# Autodesk Inventor assembly: RR_ThreeWay-A
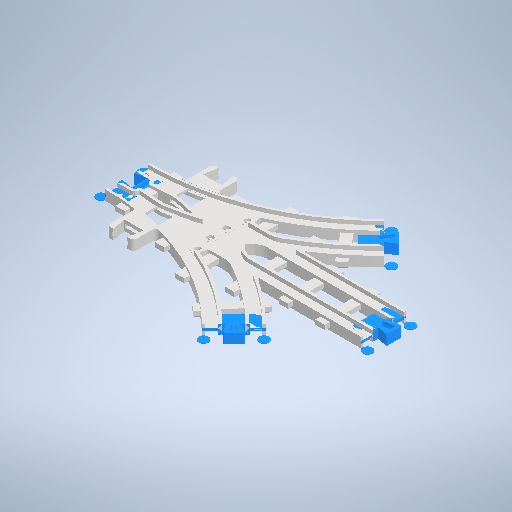
[picture p0: Inventor's stored thumbnail of the model, 512x512]
Saved by Autodesk Inventor 2025.1 (Build 291241000, 241)
## iProperties
Created: 2025-03-06
Part Number: RR_ThreeWay-A
Document SubType Name: Assembly
Designer: kumagai
Author: kumagai
## Documents named in this file (11)
- X:\Develop\CAD\PlaRails\RealRails\RR_ThreeWay.iam
- X:\Develop\CAD\PlaRails\Common\RailJointRS\FemaleDoubleSideWT.ipt
- X:\Develop\CAD\PlaRails\Common\RailJointRS.ipt
- X:\Develop\CAD\PlaRails\Common\RailJointRS\MaleDoubleSideWT.ipt
- X:\Develop\CAD\PlaRails\RealRails\RR_ThreeWay.ipt
- X:\Develop\CAD\PlaRails\RealRails\RR_ThreeWayPillow.ipt
- X:\Develop\CAD\PlaRails\RealRails\RR_ThreeWay\RR_ThreeWay-all.ipt
- RR_ThreeWay-A.iam
- RR_ThreeWay-AwoS.iam
- RR_ThreeWay-B.iam
- RR_ThreeWay-BwoS.iam
## Components (6 placed, 4 different names)
1. RR_ThreeWay-all:1 — フラッシュ:1, メイト:1, フラッシュ:2, フラッシュ:3, メイト:2, フラッシュ:4, フラッシュ:5, メイト:3, フラッシュ:6, フラッシュ:7, メイト:4, フラッシュ:8
2. FemaleDoubleSideWT:1 — フラッシュ:1, メイト:1, フラッシュ:2
3. MaleDoubleSideWT:2 — フラッシュ:3, メイト:2, フラッシュ:4
4. MaleDoubleSideWT:3 — フラッシュ:5, メイト:3, フラッシュ:6
5. RR_ThreeWayPillow:1
6. MaleDoubleSideWT:4 — フラッシュ:7, メイト:4, フラッシュ:8
## Relationships (12: Flush 8, Mate 4)
- フラッシュ:1 [Flush]: RR_ThreeWay-all:1 ↔ FemaleDoubleSideWT:1
- メイト:1 [Mate]: RR_ThreeWay-all:1 ↔ FemaleDoubleSideWT:1
- フラッシュ:2 [Flush]: RR_ThreeWay-all:1 ↔ FemaleDoubleSideWT:1
- フラッシュ:3 [Flush]: RR_ThreeWay-all:1 ↔ MaleDoubleSideWT:2
- メイト:2 [Mate]: RR_ThreeWay-all:1 ↔ MaleDoubleSideWT:2
- フラッシュ:4 [Flush]: RR_ThreeWay-all:1 ↔ MaleDoubleSideWT:2
- フラッシュ:5 [Flush]: RR_ThreeWay-all:1 ↔ MaleDoubleSideWT:3
- メイト:3 [Mate]: RR_ThreeWay-all:1 ↔ MaleDoubleSideWT:3
- フラッシュ:6 [Flush]: RR_ThreeWay-all:1 ↔ MaleDoubleSideWT:3
- フラッシュ:7 [Flush]: RR_ThreeWay-all:1 ↔ MaleDoubleSideWT:4
- メイト:4 [Mate]: RR_ThreeWay-all:1 ↔ MaleDoubleSideWT:4
- フラッシュ:8 [Flush]: RR_ThreeWay-all:1 ↔ MaleDoubleSideWT:4
